# Autodesk Inventor assembly: Top Rail assy
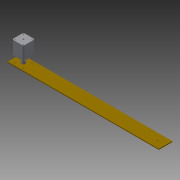
[picture p0: Inventor's stored thumbnail of the model, 180x180]
Saved by Autodesk Inventor 2013 (Build 170138000, 138)
## iProperties
Created: 2017-01-25
Part Number: Top Rail assy
Document SubType Name: Assembly
Designer: Herman de Vries
Author: Herman de Vries
## Documents named in this file (4)
- D:\Projects\Inventor\PaintBoid_2\Top Rail assy.iam
- D:\Projects\Inventor\PaintBoid_2\Top Rail.ipt
- D:\Projects\Inventor\PaintBoid_2\NEMA42.ipt
- D:\Projects\Inventor\PaintBoid_2\gear belt.ipt
## Components (3 placed, 3 different names)
1. Top Rail:1 — Mate:1, Mate:2, Mate:3
2. NEMA42:1 — Insert:1, Mate:1, Mate:2, Mate:3
3. gear belt:1 — Insert:1
## Relationships (4: Mate 3, Insert 1)
- Insert:1: NEMA42:1 ↔ gear belt:1
- Mate:1 (26 mm): Top Rail:1 ↔ NEMA42:1
- Mate:2: Top Rail:1 ↔ NEMA42:1
- Mate:3: Top Rail:1 ↔ NEMA42:1
